# Autodesk Inventor assembly: 61300811121 (rev1)
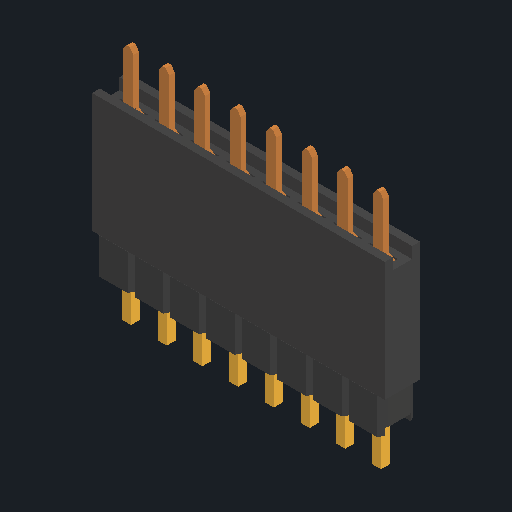
[picture p0: Inventor's stored thumbnail of the model, 512x512]
Saved by Autodesk Inventor 2022 (Build 260153000, 153)
## iProperties
Company: Unknown
Created: 2021-04-15
Part Number: 61300811121 (rev1)
Description: Unknown
Document SubType Name: Assembly
Designer: dvorakj
Authority: Unknown
Sending System: Solid Edge
Preprocessor: ST-DEVELOPER v16.7
Title: 61300811121
Author: Unknown
## Documents named in this file (4)
- C:\Users\dvorakj\Documents\Inventor\Bakalarka\Clicks\Pin Header\61300811121 (rev1).iam
- C:\Users\dvorakj\Documents\Inventor\Bakalarka\Clicks\Pin Header\61300811121.ipt
- C:\Users\dvorakj\Documents\Inventor\Bakalarka\Clicks\Pin Header\6130xx11121_PIN.ipt
- C:\Users\dvorakj\Documents\Inventor\Bakalarka\Common\Header\61300811821 (rev1).iam
## Components (10 placed, 3 different names)
1. 61300811121 — Mate:1, Angle:1, Mate:2
2. 6130xx11121_PIN
3. 6130xx11121_PIN:1
4. 6130xx11121_PIN:2
5. 6130xx11121_PIN:3
6. 6130xx11121_PIN:4
7. 6130xx11121_PIN:5
8. 6130xx11121_PIN:6
9. 6130xx11121_PIN:7
10. 61300811821 (rev1):1 [sub-assembly] — Mate:1, Angle:1, Mate:2
## Relationships (3: Mate 2, Angle 1)
- Mate:1: 61300811121 ↔ 61300811821 (rev1):1
- Angle:1 (0 deg): 61300811121 ↔ 61300811821 (rev1):1
- Mate:2: 61300811121 ↔ 61300811821 (rev1):1
